# Autodesk Inventor assembly: Animação Morsa Inventor Studio
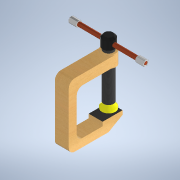
[picture p0: Inventor's stored thumbnail of the model, 180x180]
Saved by Autodesk Inventor 2021 (Build 250183000, 183)
## iProperties
Created: 2021-05-20
Part Number: Animação Morsa Inventor Studio
Document SubType Name: Assembly
Designer: rubia
Author: rubia
## Documents named in this file (6)
- C:\Users\rubia\OneDrive\Documentos\Inventor\Rubia_ASR10\Animação Morsa Inventor Studio.iam
- C:\Users\rubia\OneDrive\Documentos\Inventor\Rubia_ASR10\Apoio da Haste.ipt
- C:\Users\rubia\OneDrive\Documentos\Inventor\Rubia_ASR10\Apoio da Morsa.ipt
- C:\Users\rubia\OneDrive\Documentos\Inventor\Rubia_ASR10\Corpo da Morsa.ipt
- C:\Users\rubia\OneDrive\Documentos\Inventor\Rubia_ASR10\Haste da Morsa.ipt
- C:\Users\rubia\OneDrive\Documentos\Inventor\Rubia_ASR10\Prisioneiro.ipt
## Components (6 placed, 5 different names)
1. Apoio da Haste:1 — Coincidente:6, Coincidente:7
2. Apoio da Morsa:1 — Coincidente:8, Coincidente:9, Coincidente:10
3. Corpo da Morsa:1 — Coincidente:1, Coincidente:10
4. Haste da Morsa:1 — Coincidente:2, Coincidente:3, Coincidente:4, Coincidente:5, Coincidente:6, Coincidente:7
5. Prisioneiro:1 — Coincidente:1, Coincidente:2, Coincidente:3, Coincidente:8, Coincidente:9
6. Apoio da Haste:2 — Coincidente:4, Coincidente:5
## Relationships (10: Mate 10)
- Coincidente:1 [Mate]: Corpo da Morsa:1 ↔ Prisioneiro:1
- Coincidente:2 [Mate]: Haste da Morsa:1 ↔ Prisioneiro:1
- Coincidente:3 [Mate] (-150 mm): Haste da Morsa:1 ↔ Prisioneiro:1
- Coincidente:4 [Mate]: Haste da Morsa:1 ↔ Apoio da Haste:2
- Coincidente:5 [Mate]: Haste da Morsa:1 ↔ Apoio da Haste:2
- Coincidente:6 [Mate]: Apoio da Haste:1 ↔ Haste da Morsa:1
- Coincidente:7 [Mate]: Apoio da Haste:1 ↔ Haste da Morsa:1
- Coincidente:8 [Mate]: Apoio da Morsa:1 ↔ Prisioneiro:1
- Coincidente:9 [Mate]: Apoio da Morsa:1 ↔ Prisioneiro:1
- Coincidente:10 [Mate] (10 mm): Apoio da Morsa:1 ↔ Corpo da Morsa:1
